# Autodesk Inventor assembly: Assembly
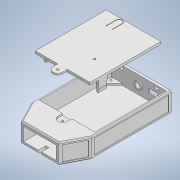
[picture p0: Inventor's stored thumbnail of the model, 180x180]
Saved by Autodesk Inventor 2021 (Build 250183000, 183)
## iProperties
Created: 2021-04-28
Part Number: Assembly
Document SubType Name: Assembly
Designer: mista
Author: mista
## Documents named in this file (3)
- C:\Users\mista\Documents\GitHub\node-a\Inventor\housing.v.2.1\Assembly.iam
- C:\Users\mista\Documents\GitHub\node-a\Inventor\housing.v.2.1\Bottom.ipt
- C:\Users\mista\Documents\GitHub\node-a\Inventor\housing.v.2.1\Top.ipt
## Components (2 placed, 2 different names)
1. Bottom:1 — Mate:1, Flush:1, Mate:2
2. Top:1 — Mate:1, Flush:1, Mate:2
## Relationships (3: Mate 2, Flush 1)
- Mate:1 (0.3302 mm): Bottom:1 ↔ Top:1
- Flush:1: Bottom:1 ↔ Top:1
- Mate:2 (0.3302 mm): Bottom:1 ↔ Top:1
